# Autodesk Inventor assembly: wrist
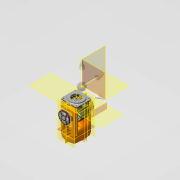
[picture p0: Inventor's stored thumbnail of the model, 180x180]
Saved by Autodesk Inventor 2016 (Build 200138000, 138)
## iProperties
Created: 2015-01-19
Part Number: wrist
Document SubType Name: Assembly
Designer: 4ndreas
Author: 4ndreas
## Documents named in this file (12)
- C:\Users\4ndreas\Documents\Inventor\RobotARM v2\v3\wrist.iam
- C:\Users\4ndreas\Documents\Inventor\RobotARM v2\v2\RotaryArm_orange.ipt
- C:\Users\4ndreas\Documents\Inventor\RobotARM v2\v2\conrad_getriebe_motor.ipt
- C:\Users\4ndreas\Documents\Inventor\RobotARM v2\v2\foreArm.ipt
- C:\Users\4ndreas\Documents\Inventor\RobotARM v2\v2\wrist_2\Konstruktions-Assistent\Stirnräder1.iam
- C:\Users\4ndreas\Documents\Inventor\RobotARM v2\servo.ipt
- C:\Users\4ndreas\Documents\Inventor\RobotARM v2\v2\encoder.iam
- C:\Users\4ndreas\Documents\Inventor\RobotARM v2\70mmkugellager.ipt
- C:\Users\4ndreas\Documents\Inventor\Gripper\3-Finger Gripper\flanschadapter.ipt
- C:\Users\4ndreas\Documents\Inventor\RobotARM v2\v2\wirstgear.ipt
- C:\Users\4ndreas\Documents\Inventor\Content Center Files\R2014\de-DE\DIN BEARING(1)\DIN 625 SKF - SKF 626.ipt
- C:\Users\4ndreas\Documents\Inventor\Content Center Files\R2014\de-DE\DIN 931-1\DIN 931-1 - M6 x 35.ipt
## Components (13 placed, 11 different names)
1. RotaryArm_orange:1 — Passend:2, Winkel:1, Passend:7, Passend:8, Passend:11, Passend:12, Passend:17, Passend:18, Winkel:4, Passend:30, Passend:31, Passend:32, Passend:34, Passend:35, Passend:39, Passend:40
2. conrad_getriebe_motor:1 — Passend:1, Passend:3, Passend:4
3. foreArm:1 — Passend:7, Passend:8, Fluchtend:2, Fluchtend:3, Passend:14, Passend:15, Passend:16, Passend:22, Winkel:2, Winkel:4, Fluchtend:6, Fluchtend:7, Passend:42
4. Stirnräder:1 [sub-assembly] — Passend:10, Passend:11, Fluchtend:2, Fluchtend:3
5. servo:1 — Passend:13, Passend:14, Passend:16
6. encoder:1 [sub-assembly] — Passend:17, Passend:18, Passend:31
7. 70mmkugellager:1 — Passend:22, Winkel:2, Passend:27, Passend:28, Passend:41, Passend:42
8. flanschadapter:1 — Passend:27, Passend:28, Passend:41, Fluchtend:7
9. wirstgear:1 — Passend:30, Fluchtend:6
10. encoder:2 [sub-assembly] — Passend:38, Passend:39, Passend:40
11. DIN 625 SKF 626:1 — Passend:33, Passend:35
12. DIN 625 SKF 626:2 — Passend:32, Passend:33, Passend:34, Passend:36, Passend:37
13. DIN 931-1 - ersetzt durch DIN EN 24014 M6 x 35:1 — Passend:36, Passend:37, Passend:38
## Relationships (40: Mate 33, Flush 4, Angle 3)
- Passend:1 [Mate]: conrad_getriebe_motor:1
- Passend:2 [Mate]: RotaryArm_orange:1
- Passend:3 [Mate]: conrad_getriebe_motor:1
- Passend:4 [Mate]: conrad_getriebe_motor:1
- Passend:5 [Mate]
- Passend:6 [Mate]
- Winkel:1 [Angle] (0 deg): RotaryArm_orange:1
- Passend:7 [Mate]: RotaryArm_orange:1 ↔ foreArm:1
- Passend:8 [Mate] (2 mm): RotaryArm_orange:1 ↔ foreArm:1
- Passend:10 [Mate]: Stirnräder:1
- Passend:11 [Mate]: RotaryArm_orange:1 ↔ Stirnräder:1
- Fluchtend:2 [Flush]: foreArm:1 ↔ Stirnräder:1
- Fluchtend:3 [Flush]: foreArm:1 ↔ Stirnräder:1
- Passend:12 [Mate]: RotaryArm_orange:1
- Passend:13 [Mate]: servo:1
- Passend:14 [Mate]: foreArm:1 ↔ servo:1
- Passend:15 [Mate]: foreArm:1
- Passend:16 [Mate]: foreArm:1 ↔ servo:1
- Passend:17 [Mate]: RotaryArm_orange:1 ↔ encoder:1
- Passend:18 [Mate] (8 mm): RotaryArm_orange:1 ↔ encoder:1
- Passend:22 [Mate] (12 mm): foreArm:1 ↔ 70mmkugellager:1
- Winkel:2 [Angle] (0 deg): foreArm:1 ↔ 70mmkugellager:1
- Winkel:4 [Angle] (0 deg): RotaryArm_orange:1 ↔ foreArm:1
- Passend:27 [Mate]: 70mmkugellager:1 ↔ flanschadapter:1
- Passend:28 [Mate]: 70mmkugellager:1 ↔ flanschadapter:1
- Passend:30 [Mate]: RotaryArm_orange:1 ↔ wirstgear:1
- Fluchtend:6 [Flush]: foreArm:1 ↔ wirstgear:1
- Passend:31 [Mate]: RotaryArm_orange:1 ↔ encoder:1
- Passend:32 [Mate]: RotaryArm_orange:1 ↔ DIN 625 SKF 626:2
- Passend:33 [Mate]: DIN 625 SKF 626:1 ↔ DIN 625 SKF 626:2
- Passend:34 [Mate]: RotaryArm_orange:1 ↔ DIN 625 SKF 626:2
- Passend:35 [Mate]: RotaryArm_orange:1 ↔ DIN 625 SKF 626:1
- Passend:36 [Mate]: DIN 625 SKF 626:2 ↔ DIN 931-1 - ersetzt durch DIN EN 24014 M6 x 35:1
- Passend:37 [Mate]: DIN 625 SKF 626:2 ↔ DIN 931-1 - ersetzt durch DIN EN 24014 M6 x 35:1
- Passend:38 [Mate] (2 mm): encoder:2 ↔ DIN 931-1 - ersetzt durch DIN EN 24014 M6 x 35:1
- Passend:39 [Mate]: RotaryArm_orange:1 ↔ encoder:2
- Passend:40 [Mate]: RotaryArm_orange:1 ↔ encoder:2
- Passend:41 [Mate]: 70mmkugellager:1 ↔ flanschadapter:1
- Fluchtend:7 [Flush]: foreArm:1 ↔ flanschadapter:1
- Passend:42 [Mate]: foreArm:1 ↔ 70mmkugellager:1
